# Autodesk Inventor assembly: OZ600Receiver
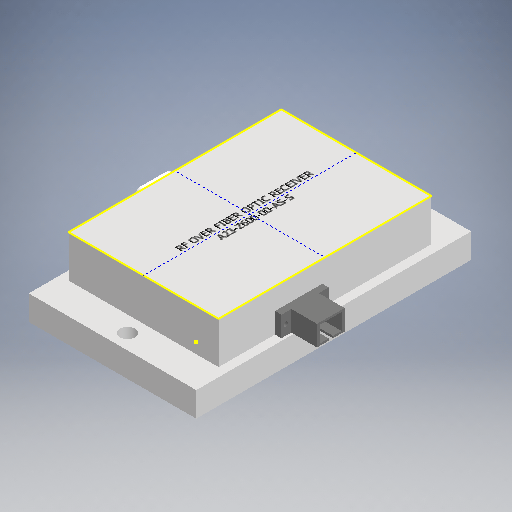
[picture p0: Inventor's stored thumbnail of the model, 512x512]
Saved by Autodesk Inventor 2025.3 (Build 293356000, 356)
## iProperties
Created: 2025-10-16
Part Number: OZ600Receiver
Document SubType Name: Assembly
Designer: sonata
Author: sonata
## Documents named in this file (5)
- D:\crush\RFoF\OZ600Receiver.iam
- D:\crush\RFoF\ReceiverBox.ipt
- D:\crush\RFoF\DB 9 Male\DB 9 Male\DB 9 Male.iam
- D:\crush\RFoF\SMA_Feedthrough.ipt
- D:\crush\RFoF\SC-adapter.ipt
## Components (4 placed, 4 different names)
1. ReceiverBox:1 — Angle:1, Angle:2, Flush:1, Flush:2, Flush:3, Flush:4, Flush:5, Tangent:1, Mate:1, Mate:2, Mate:3
2. DB 9 Male:1 [sub-assembly] — Angle:1, Angle:2, Flush:1, Flush:2, Flush:3
3. SMA_Feedthrough:1 — Flush:4, Flush:5, Tangent:1
4. SC-adapter:1 — Mate:1, Mate:2, Mate:3
## Relationships (11: Flush 5, Mate 3, Angle 2, Tangent 1)
- Angle:1 (90 deg): ReceiverBox:1 ↔ DB 9 Male:1
- Angle:2 (90 deg): ReceiverBox:1 ↔ DB 9 Male:1
- Flush:1 (-3.3528 mm): ReceiverBox:1 ↔ DB 9 Male:1
- Flush:2 (33.274 mm): ReceiverBox:1 ↔ DB 9 Male:1
- Flush:3 (5.7404 mm): ReceiverBox:1 ↔ DB 9 Male:1
- Flush:4 (-2.3114 mm): ReceiverBox:1 ↔ SMA_Feedthrough:1
- Flush:5 (11.7602 mm): ReceiverBox:1 ↔ SMA_Feedthrough:1
- Tangent:1 (6.3754 mm): ReceiverBox:1 ↔ SMA_Feedthrough:1
- Mate:1: ReceiverBox:1 ↔ SC-adapter:1
- Mate:2: ReceiverBox:1 ↔ SC-adapter:1
- Mate:3 (-48.26 mm): ReceiverBox:1 ↔ SC-adapter:1
## Named parameters: Finish1_Area = 24.6742, Finish2_Area = 24.6742
note: some values were not read from the file. Shown as the stored number, unit unknown: "Finish1_Area", "Finish2_Area".
